# Autodesk Inventor assembly: FanAssembly
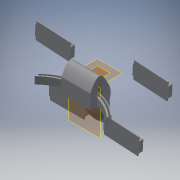
[picture p0: Inventor's stored thumbnail of the model, 180x180]
Saved by Autodesk Inventor 2016 (Build 200138000, 138)
## iProperties
Created: 2016-08-18
Part Number: FanAssembly
Document SubType Name: Assembly
Designer: yash
Author: yash
## Documents named in this file (6)
- C:\Users\yash\Documents\GitHub\ClipFanHat\FanAssembly.iam
- C:\Users\yash\Documents\GitHub\ClipFanHat\FanLip.ipt
- C:\Users\yash\Documents\GitHub\ClipFanHat\Vent.ipt
- C:\Users\yash\Documents\GitHub\ClipFanHat\Clip.ipt
- C:\Users\yash\Documents\GitHub\ClipFanHat\ClipBottom.ipt
- C:\Users\yash\Documents\GitHub\ClipFanHat\PanelHolder.ipt
## Components (8 placed, 5 different names)
1. FanLip:1 — Insert:1, Mate:5, Mate:6, Mate:7
2. Vent:1 — Insert:1, Mate:1, Mate:2, Mate:3
3. Clip:1 — Flush:1, Flush:2, Flush:3, Flush:4, Mate:4
4. ClipBottom:1 — Mate:1, Mate:2, Mate:3, Flush:1, Flush:2, Flush:3, Flush:4, Mate:4
5. PanelHolder:1
6. PanelHolder:2
7. PanelHolder:3
8. PanelHolder:4 — Mate:5, Mate:6, Mate:7
## Relationships (12: Mate 7, Flush 4, Insert 1)
- Insert:1: FanLip:1 ↔ Vent:1
- Mate:1: Vent:1 ↔ ClipBottom:1
- Mate:2: Vent:1 ↔ ClipBottom:1
- Mate:3: Vent:1 ↔ ClipBottom:1
- Flush:1: Clip:1 ↔ ClipBottom:1
- Flush:2: Clip:1 ↔ ClipBottom:1
- Flush:3: Clip:1 ↔ ClipBottom:1
- Flush:4: Clip:1 ↔ ClipBottom:1
- Mate:4 (3.175 mm): Clip:1 ↔ ClipBottom:1
- Mate:5: FanLip:1 ↔ PanelHolder:4
- Mate:6: FanLip:1 ↔ PanelHolder:4
- Mate:7: FanLip:1 ↔ PanelHolder:4
